# Autodesk Inventor assembly: IN-12_Nixie_Board_Zusammenbau
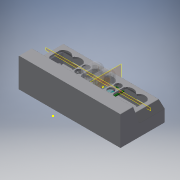
[picture p0: Inventor's stored thumbnail of the model, 180x180]
Saved by Autodesk Inventor 2019 (Build 230136000, 136)
## iProperties
Created: 2019-11-06
Part Number: IN-12_Nixie_Board_Zusammenbau
Material: Generisch
Document SubType Name: Assembly
Designer: grubi
Author: grubi
## Documents named in this file (4)
- \\diskstation\home\NixieBaugruppe\IN-12_Nixie_Board_Zusammenbau.iam
- \\diskstation\home\NixieBaugruppe\Gehaeuse_IN12_V1.1.ipt
- \\diskstation\home\NixieBaugruppe\IN-12_Nixie_Board.iam
- \\diskstation\home\NixieBaugruppe\Gehaeuse_IN12_Rueckwand_V1.1.ipt
## Components (3 placed, 3 different names)
1. Gehaeuse_IN12_V1.1:1 — Passend:1, Fluchtend:1, Passend:2, Passend:3, Passend:4
2. IN-12_Nixie_Board:1 [sub-assembly] — Passend:1, Fluchtend:1, Passend:2
3. Gehaeuse_IN12_Rueckwand_V1.1:1 — Passend:3, Passend:4
## Relationships (5: Mate 4, Flush 1)
- Passend:1 [Mate]: Gehaeuse_IN12_V1.1:1 ↔ IN-12_Nixie_Board:1
- Fluchtend:1 [Flush] (-15 mm): Gehaeuse_IN12_V1.1:1 ↔ IN-12_Nixie_Board:1
- Passend:2 [Mate]: Gehaeuse_IN12_V1.1:1 ↔ IN-12_Nixie_Board:1
- Passend:3 [Mate]: Gehaeuse_IN12_V1.1:1 ↔ Gehaeuse_IN12_Rueckwand_V1.1:1
- Passend:4 [Mate]: Gehaeuse_IN12_V1.1:1 ↔ Gehaeuse_IN12_Rueckwand_V1.1:1
